# Autodesk Inventor assembly: pillartop_testasm
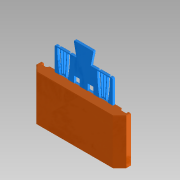
[picture p0: Inventor's stored thumbnail of the model, 180x180]
Saved by Autodesk Inventor 2021 (Build 250183000, 183)
## iProperties
Created: 2021-03-10
Part Number: pillartop_testasm
Document SubType Name: Assembly
Designer: kumagai
Author: kumagai
## Documents named in this file (3)
- X:\Develop\CAD\PlaRails\ViaductPillar\pillartop_testasm.iam
- X:\Develop\CAD\PlaRails\ViaductPillar\PillarTopVD.ipt
- X:\Develop\CAD\PlaRails\RailUnitBase.ipt
## Components (2 placed, 2 different names)
1. PillarTopVD:1 — メイト:1, メイト:2
2. RailUnitBase:1 — メイト:1, メイト:2
## Relationships (2: Mate 2)
- メイト:1 [Mate]: PillarTopVD:1 ↔ RailUnitBase:1
- メイト:2 [Mate]: PillarTopVD:1 ↔ RailUnitBase:1
